# Autodesk Inventor assembly: Assembly3
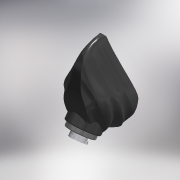
[picture p0: Inventor's stored thumbnail of the model, 180x180]
Saved by Autodesk Inventor 2021 (Build 250183000, 183)
## iProperties
Created: 2020-06-04
Part Number: Assembly3
Document SubType Name: Assembly
Designer: Derm
Author: Derm
## Documents named in this file (7)
- C:\Users\Derm\n95\v5\Assembly3.iam
- C:\Users\Derm\n95\v5\moldedBody.ipt
- C:\Users\Derm\n95\v5\3dpBayonetteMountV1Fastener.ipt
- C:\Users\Derm\n95\v5\3dpBayonetteMountV2.ipt
- C:\Users\Derm\n95\v5\Head_Dummy_DiscoverThat.ipt
- C:\Users\Derm\n95\v5\strap.ipt
- C:\Users\Derm\n95\v6\maskBody.ipt
## Components (6 placed, 6 different names)
1. moldedBody:1 — Mate:1, Mate:2, Mate:4, Mate:5, Flush:1
2. 3dpBayonetteMountV2:1 — Mate:1, Mate:2, Mate:3, Angle:1
3. 3dpBayonetteMountV1Fastener:1 — Mate:3, Mate:4, Mate:5
4. Head_Dummy_DiscoverThat:1
5. strap:1 — Flush:1
6. maskBody:1
## Relationships (7: Mate 5, Angle 1, Flush 1)
- Mate:1: moldedBody:1 ↔ 3dpBayonetteMountV2:1
- Mate:2: moldedBody:1 ↔ 3dpBayonetteMountV2:1
- Mate:3: 3dpBayonetteMountV2:1 ↔ 3dpBayonetteMountV1Fastener:1
- Mate:4: moldedBody:1 ↔ 3dpBayonetteMountV1Fastener:1
- Mate:5: moldedBody:1 ↔ 3dpBayonetteMountV1Fastener:1
- Angle:1 (0 deg): 3dpBayonetteMountV2:1
- Flush:1: moldedBody:1 ↔ strap:1
